# Autodesk Inventor assembly: Desogm Traomomg 2_Gearboxes_Exercise 2
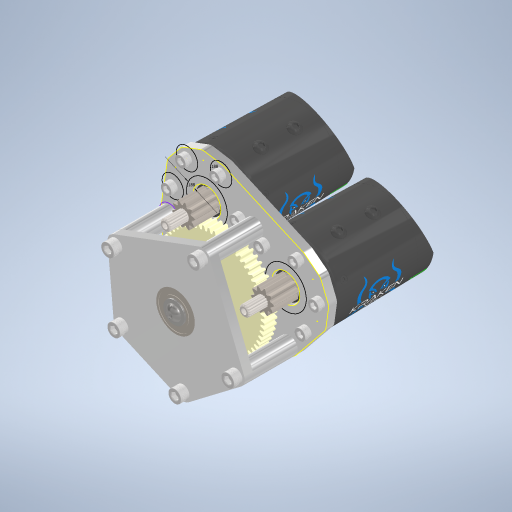
[picture p0: Inventor's stored thumbnail of the model, 512x512]
Saved by Autodesk Inventor 2024 (Build 280153000, 153)
## iProperties
Created: 2024-11-17
Part Number: Desogm Traomomg 2_Gearboxes_Exercise 2
Document SubType Name: Assembly
Designer: Danielle
Author: Danielle
## Documents named in this file (15)
- C:\Users\micha\OneDrive\Documents\GitHub\1622-2024-Assignments\Danielle\gearbox 2\Design Training 2_Gearboxes_Exercise 2.iam
- C:\Users\micha\OneDrive\Documents\GitHub\1622-2024-Assignments\Danielle\gearbox 2\gearbox 2 stuff\BottomPlate_Gearboxes_2_Exercise_2.ipt
- C:\Users\micha\OneDrive\Documents\GitHub\1622-2024-Assignments\Danielle\gearbox 2\gearbox 2 stuff\TopPlate_Gearboxes_2_Exercise_2.ipt
- C:\Users\micha\OneDrive\Documents\GitHub\1622-2024-Assignments\Danielle\gearbox 2\gearbox 2 stuff\WCP-0940\WCP-0940.ipt
- C:\Users\micha\OneDrive\Documents\GitHub\1622-2024-Assignments\Danielle\gearbox 2\gearbox 2 stuff\WCP-1008\WCP-1008.ipt
- C:\Users\micha\OneDrive\Documents\GitHub\1622-2024-Assignments\Danielle\gearbox 2\gearbox 2 stuff\WCP-0720\WCP-0720.ipt
- C:\Users\micha\OneDrive\Documents\GitHub\1622-2024-Assignments\Danielle\gearbox 2\gearbox 2 stuff\91251A342_Black-Oxide Alloy Steel Socket Head Screw\91251A342_Black-Oxide Alloy Steel Socket Head Screw.ipt
- C:\Users\micha\OneDrive\Documents\GitHub\1622-2024-Assignments\Danielle\gearbox 2\gearbox 2 stuff\WCP-0783 (2)\WCP-0783 (2).ipt
- C:\Users\micha\OneDrive\Documents\GitHub\1622-2024-Assignments\Danielle\gearbox 2\gearbox 2 stuff\91251A537_Black-Oxide Alloy Steel Socket Head Screw\91251A537_Black-Oxide Alloy Steel Socket Head Screw.ipt
- C:\Users\micha\OneDrive\Documents\GitHub\1622-2024-Assignments\COTS Library\Fasteners\Washers\COTS_90107A029_0.25in_316 Stainless Steel Washer.ipt
- C:\Users\micha\OneDrive\Documents\GitHub\1622-2024-Assignments\Danielle\gearbox 2\gearbox 2 stuff\WCP-0756\WCP-0756.ipt
- C:\Users\micha\OneDrive\Documents\GitHub\1622-2024-Assignments\Danielle\gearbox 2\gearbox 2 stuff\spacer.ipt
- C:\Users\micha\OneDrive\Documents\GitHub\1622-2024-Assignments\Danielle\gearbox 2\gearbox 2 stuff\standoff.ipt
- C:\Users\micha\OneDrive\Documents\GitHub\1622-2024-Assignments\COTS Library\Fasteners\Bolts\Button-Head\0.25-20\COTS_0.25-20_ButtonHead_0.5inlong_StainlessSteel_92949A537.ipt
- C:\Users\micha\OneDrive\Documents\GitHub\1622-2024-Assignments\Danielle\gearbox 2\gearbox 2 stuff\hexshaft_gearbox2.ipt
## Components (39 placed, 14 different names)
1. BottomPlate_Gearboxes_2_Exercise_2:1 — Mate:1, Mate:2, Mate:3, Mate:4, Mate:5, Mate:6, Mate:7, Mate:8, Mate:17, Mate:18, Mate:19, Mate:20, Mate:21, Mate:22, Mate:23, Mate:24, Mate:25, Mate:26, Mate:43, Mate:46, Mate:47, Mate:50, Mate:51, Mate:63, Mate:64, Mate:65, Mate:66, Mate:67, Mate:68, Mate:69, Mate:70, Mate:71, Mate:72
2. TopPlate_Gearboxes_2_Exercise_2:1 — Mate:1, Mate:2, Mate:27, Mate:28, Mate:44, Mate:45, Mate:48, Mate:49, Mate:52, Mate:53, Mate:54, Mate:55, Mate:56, Mate:57, Mate:58, Mate:59, Mate:60, Mate:61, Mate:62
3. WCP-0940:1 — Mate:3, Mate:4, Mate:5, Mate:13, Mate:14, Mate:15, Mate:16, Mate:35, Mate:37
4. WCP-0720:1 — Mate:31, Mate:32, Mate:38, Mate:39, Angle:2, Angle:3, Mate:42
5. 91251A342_Black-Oxide Alloy Steel Socket Head Screw:1 — Mate:13, Mate:20
6. 91251A342_Black-Oxide Alloy Steel Socket Head Screw:2 — Mate:14, Mate:22
7. 91251A342_Black-Oxide Alloy Steel Socket Head Screw:3 — Mate:15, Mate:23
8. 91251A342_Black-Oxide Alloy Steel Socket Head Screw:4 — Mate:9, Mate:18
9. 91251A342_Black-Oxide Alloy Steel Socket Head Screw:5 — Mate:16, Mate:24
10. 91251A342_Black-Oxide Alloy Steel Socket Head Screw:6 — Mate:10, Mate:17
11. 91251A342_Black-Oxide Alloy Steel Socket Head Screw:7 — Mate:12, Mate:21
12. 91251A342_Black-Oxide Alloy Steel Socket Head Screw:8 — Mate:11, Mate:19
13. WCP-0783 (2):1 — Mate:25, Mate:26, Mate:31, Mate:32, Angle:3, Mate:76
14. WCP-0783 (2):2 — Mate:27, Mate:28, Angle:4, Mate:41, Mate:73, Angle:5, Flush:1, Mate:74, Mate:75
15. 91251A537_Black-Oxide Alloy Steel Socket Head Screw:1 — Mate:65, Mate:66
16. 91251A537_Black-Oxide Alloy Steel Socket Head Screw:2 — Mate:67, Mate:68
17. 91251A537_Black-Oxide Alloy Steel Socket Head Screw:3 — Mate:69, Mate:70
18. 91251A537_Black-Oxide Alloy Steel Socket Head Screw:4 — Mate:71, Mate:72
19. 91251A537_Black-Oxide Alloy Steel Socket Head Screw:5 — Mate:63, Mate:64
20. COTS_90107A029_0.25in_316 Stainless Steel Washer:1 — Mate:74, Mate:75, Mate:81
21. COTS_90107A029_0.25in_316 Stainless Steel Washer:2 — Mate:76, Mate:77, Mate:79
22. WCP-0940:2 — Mate:6, Mate:7, Mate:8, Mate:9, Mate:10, Mate:11, Mate:12, Mate:34, Mate:36
23. WCP-1008:3 — Mate:34, Mate:36
24. WCP-1008:4 — Mate:35, Mate:37
25. WCP-0756:1 — Mate:38, Mate:40, Angle:1, Angle:4, Mate:41
26. spacer:1 — Mate:39, Mate:40, Angle:1, Angle:2, Mate:42
27. standoff:1 — Mate:47, Mate:48
28. standoff:2 — Mate:51, Mate:52
29. standoff:3 — Mate:43, Mate:44
30. standoff:4 — Mate:49, Mate:50
31. standoff:5 — Mate:45, Mate:46
32. 91251A537_Black-Oxide Alloy Steel Socket Head Screw:6 — Mate:55, Mate:56
33. 91251A537_Black-Oxide Alloy Steel Socket Head Screw:7 — Mate:57, Mate:58
34. 91251A537_Black-Oxide Alloy Steel Socket Head Screw:8 — Mate:53, Mate:54
35. 91251A537_Black-Oxide Alloy Steel Socket Head Screw:9 — Mate:61, Mate:62
36. 91251A537_Black-Oxide Alloy Steel Socket Head Screw:10 — Mate:59, Mate:60
37. COTS_0.25-20_ButtonHead_0.5inlong_StainlessSteel_92949A537:1 — Mate:78, Mate:79
38. COTS_0.25-20_ButtonHead_0.5inlong_StainlessSteel_92949A537:2 — Mate:80, Mate:81
39. hexshaft_gearbox2:1 — Mate:73, Angle:5, Flush:1, Mate:77, Mate:78, Mate:80
## Relationships (84: Mate 78, Angle 5, Flush 1)
- Mate:1: BottomPlate_Gearboxes_2_Exercise_2:1 ↔ TopPlate_Gearboxes_2_Exercise_2:1
- Mate:2: BottomPlate_Gearboxes_2_Exercise_2:1 ↔ TopPlate_Gearboxes_2_Exercise_2:1
- Mate:3: BottomPlate_Gearboxes_2_Exercise_2:1 ↔ WCP-0940:1
- Mate:4: BottomPlate_Gearboxes_2_Exercise_2:1 ↔ WCP-0940:1
- Mate:5: BottomPlate_Gearboxes_2_Exercise_2:1 ↔ WCP-0940:1
- Mate:6: BottomPlate_Gearboxes_2_Exercise_2:1 ↔ WCP-0940:2
- Mate:7: BottomPlate_Gearboxes_2_Exercise_2:1 ↔ WCP-0940:2
- Mate:8: BottomPlate_Gearboxes_2_Exercise_2:1 ↔ WCP-0940:2
- Mate:9: 91251A342_Black-Oxide Alloy Steel Socket Head Screw:4 ↔ WCP-0940:2
- Mate:10: 91251A342_Black-Oxide Alloy Steel Socket Head Screw:6 ↔ WCP-0940:2
- Mate:11: 91251A342_Black-Oxide Alloy Steel Socket Head Screw:8 ↔ WCP-0940:2
- Mate:12: 91251A342_Black-Oxide Alloy Steel Socket Head Screw:7 ↔ WCP-0940:2
- Mate:13: WCP-0940:1 ↔ 91251A342_Black-Oxide Alloy Steel Socket Head Screw:1
- Mate:14: WCP-0940:1 ↔ 91251A342_Black-Oxide Alloy Steel Socket Head Screw:2
- Mate:15: WCP-0940:1 ↔ 91251A342_Black-Oxide Alloy Steel Socket Head Screw:3
- Mate:16: WCP-0940:1 ↔ 91251A342_Black-Oxide Alloy Steel Socket Head Screw:5
- Mate:17: BottomPlate_Gearboxes_2_Exercise_2:1 ↔ 91251A342_Black-Oxide Alloy Steel Socket Head Screw:6
- Mate:18: BottomPlate_Gearboxes_2_Exercise_2:1 ↔ 91251A342_Black-Oxide Alloy Steel Socket Head Screw:4
- Mate:19: BottomPlate_Gearboxes_2_Exercise_2:1 ↔ 91251A342_Black-Oxide Alloy Steel Socket Head Screw:8
- Mate:20: BottomPlate_Gearboxes_2_Exercise_2:1 ↔ 91251A342_Black-Oxide Alloy Steel Socket Head Screw:1
- Mate:21: BottomPlate_Gearboxes_2_Exercise_2:1 ↔ 91251A342_Black-Oxide Alloy Steel Socket Head Screw:7
- Mate:22: BottomPlate_Gearboxes_2_Exercise_2:1 ↔ 91251A342_Black-Oxide Alloy Steel Socket Head Screw:2
- Mate:23: BottomPlate_Gearboxes_2_Exercise_2:1 ↔ 91251A342_Black-Oxide Alloy Steel Socket Head Screw:3
- Mate:24: BottomPlate_Gearboxes_2_Exercise_2:1 ↔ 91251A342_Black-Oxide Alloy Steel Socket Head Screw:5
- Mate:25: BottomPlate_Gearboxes_2_Exercise_2:1 ↔ WCP-0783 (2):1
- Mate:26: BottomPlate_Gearboxes_2_Exercise_2:1 ↔ WCP-0783 (2):1
- Mate:27: TopPlate_Gearboxes_2_Exercise_2:1 ↔ WCP-0783 (2):2
- Mate:28: TopPlate_Gearboxes_2_Exercise_2:1 ↔ WCP-0783 (2):2
- Mate:31: WCP-0720:1 ↔ WCP-0783 (2):1
- Mate:32: WCP-0720:1 ↔ WCP-0783 (2):1
- Mate:34: WCP-0940:2 ↔ WCP-1008:3
- Mate:35: WCP-0940:1 ↔ WCP-1008:4
- Mate:36: WCP-0940:2 ↔ WCP-1008:3
- Mate:37: WCP-0940:1 ↔ WCP-1008:4
- Mate:38: WCP-0720:1 ↔ WCP-0756:1
- Mate:39: WCP-0720:1 ↔ spacer:1
- Mate:40: WCP-0756:1 ↔ spacer:1
- Angle:1 (0 deg): WCP-0756:1 ↔ spacer:1
- Angle:2 (0 deg): WCP-0720:1 ↔ spacer:1
- Angle:3 (0 deg): WCP-0720:1 ↔ WCP-0783 (2):1
- Angle:4 (0 deg): WCP-0783 (2):2 ↔ WCP-0756:1
- Mate:41: WCP-0783 (2):2 ↔ WCP-0756:1
- Mate:42: WCP-0720:1 ↔ spacer:1
- Mate:43: BottomPlate_Gearboxes_2_Exercise_2:1 ↔ standoff:3
- Mate:44: TopPlate_Gearboxes_2_Exercise_2:1 ↔ standoff:3
- Mate:45: TopPlate_Gearboxes_2_Exercise_2:1 ↔ standoff:5
- Mate:46: BottomPlate_Gearboxes_2_Exercise_2:1 ↔ standoff:5
- Mate:47: BottomPlate_Gearboxes_2_Exercise_2:1 ↔ standoff:1
- Mate:48: TopPlate_Gearboxes_2_Exercise_2:1 ↔ standoff:1
- Mate:49: TopPlate_Gearboxes_2_Exercise_2:1 ↔ standoff:4
- Mate:50: BottomPlate_Gearboxes_2_Exercise_2:1 ↔ standoff:4
- Mate:51: BottomPlate_Gearboxes_2_Exercise_2:1 ↔ standoff:2
- Mate:52: TopPlate_Gearboxes_2_Exercise_2:1 ↔ standoff:2
- Mate:53: TopPlate_Gearboxes_2_Exercise_2:1 ↔ 91251A537_Black-Oxide Alloy Steel Socket Head Screw:8
- Mate:54: TopPlate_Gearboxes_2_Exercise_2:1 ↔ 91251A537_Black-Oxide Alloy Steel Socket Head Screw:8
- Mate:55: TopPlate_Gearboxes_2_Exercise_2:1 ↔ 91251A537_Black-Oxide Alloy Steel Socket Head Screw:6
- Mate:56: TopPlate_Gearboxes_2_Exercise_2:1 ↔ 91251A537_Black-Oxide Alloy Steel Socket Head Screw:6
- Mate:57: TopPlate_Gearboxes_2_Exercise_2:1 ↔ 91251A537_Black-Oxide Alloy Steel Socket Head Screw:7
- Mate:58: TopPlate_Gearboxes_2_Exercise_2:1 ↔ 91251A537_Black-Oxide Alloy Steel Socket Head Screw:7
- Mate:59: TopPlate_Gearboxes_2_Exercise_2:1 ↔ 91251A537_Black-Oxide Alloy Steel Socket Head Screw:10
- Mate:60: TopPlate_Gearboxes_2_Exercise_2:1 ↔ 91251A537_Black-Oxide Alloy Steel Socket Head Screw:10
- Mate:61: TopPlate_Gearboxes_2_Exercise_2:1 ↔ 91251A537_Black-Oxide Alloy Steel Socket Head Screw:9
- Mate:62: TopPlate_Gearboxes_2_Exercise_2:1 ↔ 91251A537_Black-Oxide Alloy Steel Socket Head Screw:9
- Mate:63: BottomPlate_Gearboxes_2_Exercise_2:1 ↔ 91251A537_Black-Oxide Alloy Steel Socket Head Screw:5
- Mate:64: BottomPlate_Gearboxes_2_Exercise_2:1 ↔ 91251A537_Black-Oxide Alloy Steel Socket Head Screw:5
- Mate:65: BottomPlate_Gearboxes_2_Exercise_2:1 ↔ 91251A537_Black-Oxide Alloy Steel Socket Head Screw:1
- Mate:66: BottomPlate_Gearboxes_2_Exercise_2:1 ↔ 91251A537_Black-Oxide Alloy Steel Socket Head Screw:1
- Mate:67: BottomPlate_Gearboxes_2_Exercise_2:1 ↔ 91251A537_Black-Oxide Alloy Steel Socket Head Screw:2
- Mate:68: BottomPlate_Gearboxes_2_Exercise_2:1 ↔ 91251A537_Black-Oxide Alloy Steel Socket Head Screw:2
- Mate:69: BottomPlate_Gearboxes_2_Exercise_2:1 ↔ 91251A537_Black-Oxide Alloy Steel Socket Head Screw:3
- Mate:70: BottomPlate_Gearboxes_2_Exercise_2:1 ↔ 91251A537_Black-Oxide Alloy Steel Socket Head Screw:3
- Mate:71: BottomPlate_Gearboxes_2_Exercise_2:1 ↔ 91251A537_Black-Oxide Alloy Steel Socket Head Screw:4
- Mate:72: BottomPlate_Gearboxes_2_Exercise_2:1 ↔ 91251A537_Black-Oxide Alloy Steel Socket Head Screw:4
- Mate:73: WCP-0783 (2):2 ↔ hexshaft_gearbox2:1
- Angle:5 (0 deg): WCP-0783 (2):2 ↔ hexshaft_gearbox2:1
- Flush:1: WCP-0783 (2):2 ↔ hexshaft_gearbox2:1
- Mate:74: WCP-0783 (2):2 ↔ COTS_90107A029_0.25in_316 Stainless Steel Washer:1
- Mate:75: WCP-0783 (2):2 ↔ COTS_90107A029_0.25in_316 Stainless Steel Washer:1
- Mate:76: WCP-0783 (2):1 ↔ COTS_90107A029_0.25in_316 Stainless Steel Washer:2
- Mate:77: COTS_90107A029_0.25in_316 Stainless Steel Washer:2 ↔ hexshaft_gearbox2:1
- Mate:78: COTS_0.25-20_ButtonHead_0.5inlong_StainlessSteel_92949A537:1 ↔ hexshaft_gearbox2:1
- Mate:79: COTS_90107A029_0.25in_316 Stainless Steel Washer:2 ↔ COTS_0.25-20_ButtonHead_0.5inlong_StainlessSteel_92949A537:1
- Mate:80: COTS_0.25-20_ButtonHead_0.5inlong_StainlessSteel_92949A537:2 ↔ hexshaft_gearbox2:1
- Mate:81: COTS_90107A029_0.25in_316 Stainless Steel Washer:1 ↔ COTS_0.25-20_ButtonHead_0.5inlong_StainlessSteel_92949A537:2
